# Autodesk Inventor assembly: new pulley plate lineup test
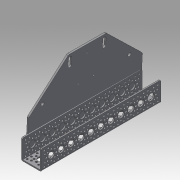
[picture p0: Inventor's stored thumbnail of the model, 180x180]
Saved by Autodesk Inventor 2016 (Build 200138000, 138)
## iProperties
Created: 2015-12-05
Part Number: new pulley plate lineup test
Document SubType Name: Assembly
Designer: Delta
Author: Delta
## Documents named in this file (3)
- C:\Robotics\CAD\2015-16\custom cad parts\new pulley plate lineup test.iam
- C:\Robotics\CAD\2015-16\COTSParts\Actobotics\585 parts\585450.ipt
- C:\Robotics\CAD\2015-16\custom cad parts\new pulley plate-v1.ipt
## Components (2 placed, 2 different names)
1. 585450:1 — Mate:1, Mate:2
2. new pulley plate-v1:1 — Mate:1, Mate:2
## Relationships (2: Mate 2)
- Mate:1: 585450:1 ↔ new pulley plate-v1:1
- Mate:2: 585450:1 ↔ new pulley plate-v1:1
